# Autodesk Inventor assembly: McCrea_car_walle
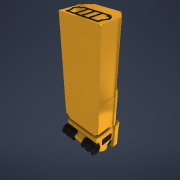
[picture p0: Inventor's stored thumbnail of the model, 180x180]
Saved by Autodesk Inventor 2022 (Build 260153000, 153)
## iProperties
Created: 2022-02-07
Part Number: McCrea_car_walle
Document SubType Name: Assembly
Designer: MatusBarany
Author: MatusBarany
## Documents named in this file (5)
- C:\Users\MatusBarany\Documents\Inventor\wall-e\assembly\McCrea_car_walle.iam
- C:\Users\MatusBarany\Documents\Inventor\wall-e\matus\electronic truck\McCrea_front_walle.ipt
- C:\Users\MatusBarany\Documents\Inventor\wall-e\matus\electronic truck\McCrea_front_wheel_walle.ipt
- C:\Users\MatusBarany\Documents\Inventor\wall-e\matus\electronic truck\McCrea_roof_walle.ipt
- C:\Users\MatusBarany\Documents\Inventor\wall-e\lukas\McCrea_Auto_walle.ipt
## Components (7 placed, 4 different names)
1. McCrea_front_walle:1 — Mate:1, Mate:2, Flush:1, Rigid:1, Rigid:3
2. McCrea_front_wheel_walle:1 — Rigid:2
3. McCrea_roof_walle:1 — Mate:1, Mate:2, Flush:1, Mate:3, Flush:2, Flush:3
4. McCrea_front_wheel_walle:2 — Rigid:1, Rigid:2
5. McCrea_front_wheel_walle:3 — Rigid:3, Rotational:1
6. McCrea_front_wheel_walle:4 — Rotational:1
7. McCrea_Auto_walle:1 — Mate:3, Flush:2, Flush:3
## Relationships (10: Mate 3, Flush 3, WeldJoint 3, RevoluteJoint 1)
- Mate:1: McCrea_front_walle:1 ↔ McCrea_roof_walle:1
- Mate:2: McCrea_front_walle:1 ↔ McCrea_roof_walle:1
- Flush:1: McCrea_front_walle:1 ↔ McCrea_roof_walle:1
- Rigid:1 [WeldJoint]: McCrea_front_walle:1 ↔ McCrea_front_wheel_walle:2
- Rigid:2 [WeldJoint]: McCrea_front_wheel_walle:1 ↔ McCrea_front_wheel_walle:2
- Rigid:3 [WeldJoint]: McCrea_front_walle:1 ↔ McCrea_front_wheel_walle:3
- Rotational:1 [RevoluteJoint]: McCrea_front_wheel_walle:3 ↔ McCrea_front_wheel_walle:4
- Mate:3: McCrea_roof_walle:1 ↔ McCrea_Auto_walle:1
- Flush:2: McCrea_roof_walle:1 ↔ McCrea_Auto_walle:1
- Flush:3: McCrea_roof_walle:1 ↔ McCrea_Auto_walle:1
